# Autodesk Inventor assembly: Cable-Organizer Unit
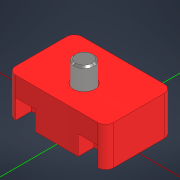
[picture p0: Inventor's stored thumbnail of the model, 180x180]
Saved by Autodesk Inventor 2022.2 (Build 262287010, 287A)
## iProperties
Created: 2022-03-23
Part Number: Cable-Organizer Unit
Document SubType Name: Assembly
Designer: sleib
Author: sleib
## Documents named in this file (3)
- C:\Users\sleib\Projekte\Voron-2\CAD\Inventor\Cable-Organizer Unit.iam
- C:\Users\sleib\Projekte\Voron-2\CAD\Inventor\Cable-Organizer.ipt
- C:\Users\sleib\Projekte\Voron-2\CAD\Inventor\M5x10 BHCS.ipt
## Components (2 placed, 2 different names)
1. Cable-Organizer:1 — Passend:1, Passend:2
2. M5x10 BHCS:1 — Passend:1, Passend:2
## Relationships (2: Mate 2)
- Passend:1 [Mate]: Cable-Organizer:1 ↔ M5x10 BHCS:1
- Passend:2 [Mate]: Cable-Organizer:1 ↔ M5x10 BHCS:1
